# Autodesk Inventor assembly: Drivair
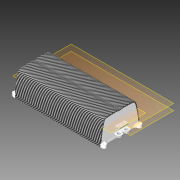
[picture p0: Inventor's stored thumbnail of the model, 180x180]
Saved by Autodesk Inventor 2016 (Build 200138000, 138)
## iProperties
Created: 2015-06-09
Part Number: Drivair
Document SubType Name: Assembly
Designer: Yann
Author: Yann
## Documents named in this file (8)
- C:\Users\Yann\Documents\GitHub\BIKAIR_CAD\Source\Powertrain_Controller\Drivair.iam
- C:\Users\Yann\Documents\GitHub\BIKAIR_CAD\Source\Powertrain_Controller\Heatsink.ipt
- C:\Users\Yann\Documents\GitHub\BIKAIR_CAD\Source\Powertrain_Controller\PowerPCB.ipt
- C:\Users\Yann\Documents\GitHub\BIKAIR_CAD\Source\Powertrain_Controller\LogicPCB.ipt
- C:\Users\Yann\Documents\GitHub\BIKAIR_CAD\Source\Powertrain_Controller\HostPCB.ipt
- C:\Users\Yann\Documents\GitHub\BIKAIR_CAD\Source\Powertrain_Controller\Cover.ipt
- C:\Users\Yann\Documents\GitHub\BIKAIR_CAD\Source\Powertrain_Controller\Interface_Left_Pannel.ipt
- C:\Users\Yann\Documents\GitHub\BIKAIR_CAD\Source\Powertrain_Controller\Parameters.xlsx
## Components (6 placed, 6 different names)
1. Heatsink:1 — Flush:1, Flush:2, Flush:3, Flush:20
2. PowerPCB:1 — Flush:5, Flush:6, Flush:7
3. LogicPCB:1 — Flush:9, Flush:10, Flush:11, Flush:12
4. HostPCB:1 — Flush:13, Flush:14, Flush:15, Flush:16
5. Cover:1 — Flush:18, Mate:1, Mate:2
6. Interface_Left_Pannel:1 — Flush:19, Flush:20, Flush:21
## Relationships (22: Flush 20, Mate 2)
- Flush:1: Heatsink:1
- Flush:2: Heatsink:1
- Flush:3: Heatsink:1
- Flush:4 (1.2 mm)
- Flush:5: PowerPCB:1
- Flush:6: PowerPCB:1
- Flush:7: PowerPCB:1
- Flush:8 (11 mm)
- Flush:9: LogicPCB:1
- Flush:10: LogicPCB:1
- Flush:11: LogicPCB:1
- Flush:12 (8 mm): LogicPCB:1
- Flush:13: HostPCB:1
- Flush:14: HostPCB:1
- Flush:15: HostPCB:1
- Flush:16 (8 mm): HostPCB:1
- Flush:18: Cover:1
- Mate:1: Cover:1
- Mate:2: Cover:1
- Flush:19: Interface_Left_Pannel:1
- Flush:20: Heatsink:1 ↔ Interface_Left_Pannel:1
- Flush:21: Interface_Left_Pannel:1
## Named parameters: Heatsink_Length = 150 mm, Heatsink_Thickness = 5 mm, Heatsink_Width = 65 mm, Cover_Thickness = 2 mm, PowerPCB_Minus_Height = 1.2 mm, PowerPCB_Width = 63 mm, PowerPCB_Length = 170 mm, Interface_Thickness = 7 mm, PowerPCB_Thickness = 3 mm, PowerPCB_Plus_Height = 8 mm, LogicPCB_Width = 55 mm, LogicPCB_Thickness = 2 mm, LogicPCB_Plus_Height = 8 mm, HostPCB_Length = 130 mm, HostPCB_Width = 50 mm, HostPCB_Plus_Height = 8 mm, HostPCB_Thickness = 1.2 mm
